# Autodesk Inventor assembly: Assembly1
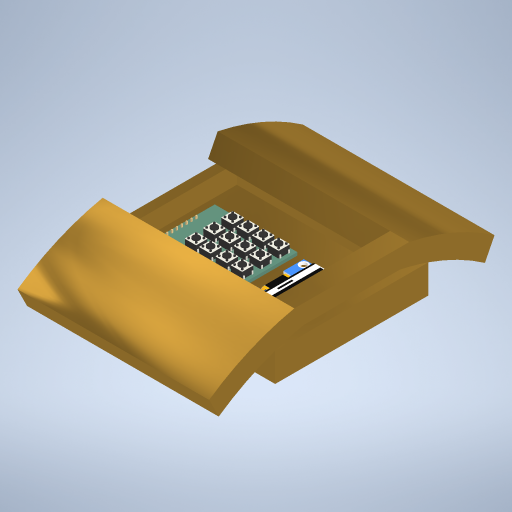
[picture p0: Inventor's stored thumbnail of the model, 512x512]
Saved by Autodesk Inventor 2024 (Build 280153000, 153)
## iProperties
Created: 2024-09-17
Part Number: Assembly1
Document SubType Name: Assembly
Designer: domko
Author: domko
## iProperties of the stored document PinHeader_1x08_P2.54mm_Vertical.iam
Created: 2024-09-17
Part Number: PinHeader_1x08_P2.54mm_Vertical
Document SubType Name: Assembly
Designer: domko
Author: domko
## iProperties of the stored document PinHeader_1x08_P254mm_Vertical.ipt
Created: 2024-09-17
Part Number: PinHeader_1x08_P254mm_Vertical
Material: Generic
Document SubType Name: Modeling
Designer: domko
Density: 1 g/cm^3
Appearance: Default
Author: domko
## iProperties of the stored document _autosave-CzlapCzlapTOP_PCB.ipt
Created: 2024-09-17
Part Number: _autosave-CzlapCzlapTOP_PCB
Material: Generic
Document SubType Name: Modeling
Designer: domko
Density: 1 g/cm^3
Appearance: Default
Author: domko
## iProperties of the stored document SW_PUSH_6mm.iam
Created: 2024-09-17
Part Number: SW_PUSH_6mm
Document SubType Name: Assembly
Designer: domko
Author: domko
## iProperties of the stored document SW_PUSH_6mm.ipt
Created: 2024-09-17
Part Number: SW_PUSH_6mm
Material: Generic
Document SubType Name: Modeling
Designer: domko
Density: 1 g/cm^3
Appearance: Default
Author: domko
## iProperties of the stored document tact_keyboard_botpins.iam
Created: 2024-07-23
Part Number: tact_keyboard 1
Description: KiCad electronic assembly
Document SubType Name: Assembly
Designer: domko
Authority: Unknown
Company: Kicad
Title: tact_keyboard.step
Author: Pcbnew
Sending System: KiCad to STEP converter
Preprocessor: Open CASCADE STEP processor 7.7
## Documents named in this file (10)
- **C:\Users\Public\Documents\Autodesk\Inventor 2024\czlapczlap_test\Assembly1.iam*LocalDocs*xAaaaabcaAaaaaaaaAaaaah2pLd*PinHeader_1x08_P2.54mm_Vertical.iam
- **C:\Users\Public\Documents\Autodesk\Inventor 2024\czlapczlap_test\Assembly1.iam*LocalDocs*xAaaaa3daAaaaaaaaAaaaaylu3g*PinHeader_1x08_P254mm_Vertical.ipt
- **C:\Users\Public\Documents\Autodesk\Inventor 2024\czlapczlap_test\Assembly1.iam*LocalDocs*xAaaaardaAaaaaaaaAaaaq1rfTc*_autosave-CzlapCzlapTOP_PCB.ipt
- **C:\Users\Public\Documents\Autodesk\Inventor 2024\czlapczlap_test\Assembly1.iam*LocalDocs*xAaaaanbaAaaaaaaaAaaaaeayGe*SW_PUSH_6mm.iam
- **C:\Users\Public\Documents\Autodesk\Inventor 2024\czlapczlap_test\Assembly1.iam*LocalDocs*xAaaaqtbaAaaaaaaaAaaaa1r5Ga*SW_PUSH_6mm.ipt
- **C:\Users\Public\Documents\Autodesk\Inventor 2024\czlapczlap_test\Assembly1.iam*LocalDocs*xAaaaqycaAaaaaaaaAaaaackkLh*tact_keyboard_botpins.iam
- C:\Users\Public\Documents\Autodesk\Inventor 2024\czlapczlap_test\Assembly1.iam
- C:\Users\Public\Documents\Autodesk\Inventor 2024\czlapczlap_test\Part1.ipt
- C:\Users\Public\Documents\Autodesk\Inventor 2024\czlapczlap_test\ER-OLEDM013-1-SPI-I2C\ER-OLEDM013-1-SPI-I2C.iam
- C:\Users\Public\Documents\Autodesk\Inventor 2024\czlapczlap_test\tact_keyboard_botpins.step
## Components (3 placed, 3 different names)
1. Part1:1 — Mate:1, Mate:2, Mate:3, Mate:4, Mate:5, Mate:6
2. ER-OLEDM013-1-SPI-I2C:2 [sub-assembly] — Mate:1, Mate:2, Mate:3
3. tact_keyboard_botpins:1 [sub-assembly] — Mate:4, Mate:5, Mate:6
## Relationships (6: Mate 6)
- Mate:1: Part1:1 ↔ ER-OLEDM013-1-SPI-I2C:2
- Mate:2: Part1:1 ↔ ER-OLEDM013-1-SPI-I2C:2
- Mate:3: Part1:1 ↔ ER-OLEDM013-1-SPI-I2C:2
- Mate:4: Part1:1 ↔ tact_keyboard_botpins:1
- Mate:5: Part1:1 ↔ tact_keyboard_botpins:1
- Mate:6: Part1:1 ↔ tact_keyboard_botpins:1
